# Autodesk Inventor assembly: Chassi
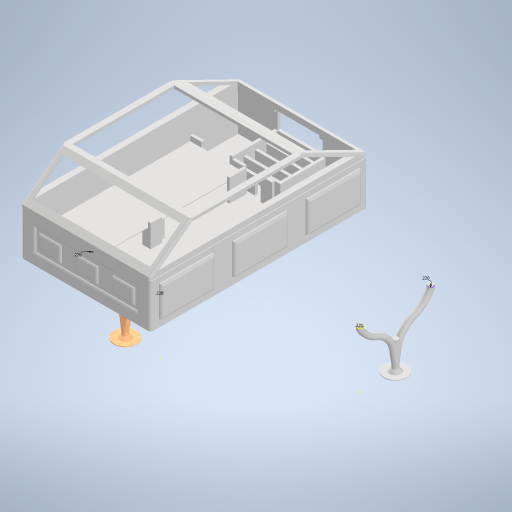
[picture p0: Inventor's stored thumbnail of the model, 512x512]
Saved by Autodesk Inventor 2023.4 (Build 274418000, 418)
## iProperties
Created: 2026-02-23
Part Number: Chassi
Document SubType Name: Assembly
Designer: 1017208
Author: 1017208
## Documents named in this file (5)
- C:\Users\1017208\OneDrive - Loudoun County Public Schools\Documents\RSEF\3DPrint\Chassis.iam
- C:\Users\1017208\OneDrive - Loudoun County Public Schools\Documents\RSEF\3DPrint\SimpleElectronicBoxV2.0.ipt
- C:\Users\1017208\OneDrive - Loudoun County Public Schools\Documents\RSEF\3DPrint\TopLid.ipt
- C:\Users\1017208\OneDrive - Loudoun County Public Schools\Documents\RSEF\3DPrint\ElevationPlate.ipt
- C:\Users\1017208\OneDrive - Loudoun County Public Schools\Documents\RSEF\3DPrint\Stands.ipt
## Components (5 placed, 4 different names)
1. SimpleElectronicBoxV2.0:1 — Rigid:1, Rigid:2, Rigid:3
2. TopLid:1 — Rigid:1
3. ElevationPlate:1 — Rigid:2
4. Stands:1 — Rigid:3
5. Stands:2
## Relationships (3: WeldJoint 3)
- Rigid:1 [WeldJoint]: SimpleElectronicBoxV2.0:1 ↔ TopLid:1
- Rigid:2 [WeldJoint]: SimpleElectronicBoxV2.0:1 ↔ ElevationPlate:1
- Rigid:3 [WeldJoint]: SimpleElectronicBoxV2.0:1 ↔ Stands:1
